# Autodesk Inventor assembly: 15102898-16-A-1000
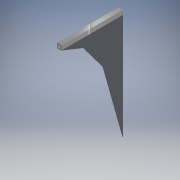
[picture p0: Inventor's stored thumbnail of the model, 180x180]
Saved by Autodesk Inventor 2017 (Build 210142000, 142)
## iProperties
Created: 2016-11-08
Part Number: 15102898-16-A-1000
Document SubType Name: Assembly
Designer: gus
Author: gus
## Documents named in this file (3)
- \\Mac\Home\Desktop\bunnybots 2016\15102898-16-Bunnybot-CAD\Bunnybot-Night_Fury\15102898-16-A-0000\15102898-16-A-1000\15102898-16-A-1000.iam
- \\Mac\Home\Desktop\bunnybots 2016\15102898-16-Bunnybot-CAD\Bunnybot-Night_Fury\15102898-16-A-0000\15102898-16-A-1000\15102898-16-P-0101.ipt
- \\Mac\Home\Desktop\bunnybots 2016\15102898-16-Bunnybot-CAD\Bunnybot-Night_Fury\15102898-16-A-0000\15102898-16-A-1000\15102898-16-P-0102.ipt
## Components (2 placed, 2 different names)
1. 15102898-16-P-0101:1 — Mate:1, Flush:1, Mate:2
2. 15102898-16-P-0102:1 — Mate:1, Flush:1, Mate:2
## Relationships (3: Mate 2, Flush 1)
- Mate:1: 15102898-16-P-0101:1 ↔ 15102898-16-P-0102:1
- Flush:1: 15102898-16-P-0101:1 ↔ 15102898-16-P-0102:1
- Mate:2: 15102898-16-P-0101:1 ↔ 15102898-16-P-0102:1
